# Autodesk Inventor assembly: Reducer_Motor_HG-KR13
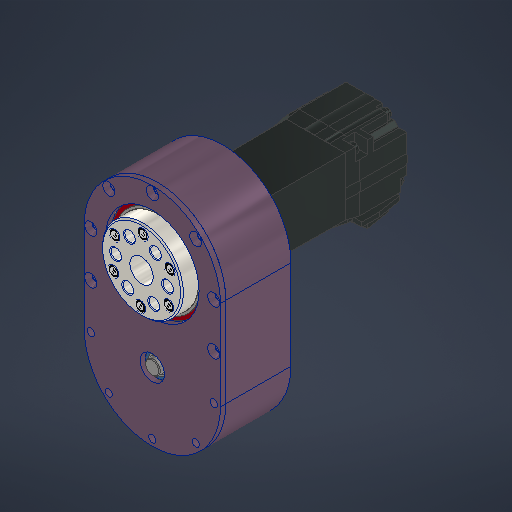
[picture p0: Inventor's stored thumbnail of the model, 512x512]
Saved by Autodesk Inventor 2026 (Build 300175000, 175)
## iProperties
Created: 2025-12-04
Part Number: Reducer_Motor_HG-KR13
Document SubType Name: Assembly
Designer: DanielFGarzon
Mass: 1257.96 g
Surface Area: 1181.01 cm^2
Volume: 298.819 cm^3
Density: 4.20977 g/cm^3
Author: DanielFGarzon
## Documents named in this file (17)
- D:\POLIMI\3RD SEMESTER\Industrial Robotics\Project\Mine\Reducer_02\Reducer_Motor_HG-KR13.iam
- D:\POLIMI\3RD SEMESTER\Industrial Robotics\Project\Mine\Reducer_02\Housing.ipt
- D:\POLIMI\3RD SEMESTER\Industrial Robotics\Project\Mine\Reducer_02\Bearing_08_16_04.ipt
- D:\POLIMI\3RD SEMESTER\Industrial Robotics\Project\Mine\Reducer_02\Bearing_08_26_08.ipt
- D:\POLIMI\3RD SEMESTER\Industrial Robotics\Project\Mine\Reducer_02\Shaft_8mm.ipt
- D:\POLIMI\3RD SEMESTER\Industrial Robotics\Project\Mine\Reducer_02\Motor_HG-KR13.ipt
- D:\POLIMI\3RD SEMESTER\Industrial Robotics\Project\Mine\Reducer_02\Washer_M8_12_0.3.ipt
- D:\POLIMI\3RD SEMESTER\Industrial Robotics\Project\Mine\Reducer_02\Pulley_3M12T_01.ipt
- D:\POLIMI\3RD SEMESTER\Industrial Robotics\Project\Mine\Reducer_02\Washer_M8_10_3.8.ipt
- D:\POLIMI\3RD SEMESTER\Industrial Robotics\Project\Mine\Reducer_02\Pulley_3M60T_01.ipt
- D:\POLIMI\3RD SEMESTER\Industrial Robotics\Project\Mine\Reducer_02\Washer_M8_14_0.5.ipt
- D:\POLIMI\3RD SEMESTER\Industrial Robotics\Project\Mine\Reducer_02\Pulley_3M12T_02.ipt
- D:\POLIMI\3RD SEMESTER\Industrial Robotics\Project\Mine\Reducer_02\Pulley_3M60T_02.ipt
- D:\POLIMI\3RD SEMESTER\Industrial Robotics\Project\Mine\Reducer_02\ActuationDisk.ipt
- D:\POLIMI\3RD SEMESTER\Industrial Robotics\Project\Mine\Reducer_02\Bearing_45_55_06.ipt
- D:\POLIMI\3RD SEMESTER\Industrial Robotics\Project\Mine\Reducer_02\Cover.ipt
- D:\POLIMI\3RD SEMESTER\Industrial Robotics\Project\Mine\Reducer_02\M3_Screw.ipt
## Components (23 placed, 16 different names)
1. Housing:1 — Mate:1, Mate:2, Flush:1, Mate:4, Mate:5, Mate:6, Mate:45
2. Bearing_08_16_04:1 — Mate:1, Mate:2, Mate:3, Mate:7
3. Bearing_08_26_08:1 — Mate:22, Mate:30, Mate:34, Mate:35
4. Shaft_8mm:1 — Mate:3, Flush:1, Mate:8, Mate:20, Mate:27, Mate:32, Mate:47
5. Motor_HG-KR13:1 — Mate:4, Mate:5, Mate:6, Mate:11, Mate:12, Mate:22, Mate:24, Mate:25, Mate:29
6. Washer_M8_12_0.3:1 — Mate:7, Mate:8, Mate:26
7. Pulley_3M12T_01:1 — Mate:23, Mate:25, Mate:28
8. Washer_M8_10_3.8:1 — Mate:11, Mate:12, Mate:23, Mate:24
9. Pulley_3M60T_01:1 — Mate:26, Mate:27, Mate:33
10. Washer_M8_14_0.5:1 — Mate:28, Mate:29, Mate:30
11. Washer_M8_14_0.5:2 — Mate:20, Mate:31, Mate:33
12. Pulley_3M12T_02:1 — Mate:31, Mate:32
13. Pulley_3M60T_02:1 — Mate:34, Mate:35, Mate:40, Mate:41, Mate:42
14. ActuationDisk:1 — Mate:40, Mate:41, Mate:42, Mate:43, Mate:44, Mate:46, Mate:50, Mate:51, Mate:52, Mate:53, Mate:54, Mate:55, Flush:2, Flush:3, Flush:4, Flush:5, Flush:6, Flush:7
15. Bearing_45_55_06:1 — Mate:43, Mate:44
16. Cover:1 — Mate:45, Mate:46, Mate:47, Mate:48, Mate:49
17. Bearing_08_16_04:3 — Mate:48, Mate:49
18. M3_Screw:1 — Mate:51, Flush:3
19. M3_Screw:2 — Mate:55, Flush:6
20. M3_Screw:3 — Mate:54, Flush:5
21. M3_Screw:4 — Mate:50, Flush:2
22. M3_Screw:5 — Mate:52, Flush:4
23. M3_Screw:6 — Mate:53, Flush:7
## Relationships (48: Mate 41, Flush 7)
- Mate:1: Housing:1 ↔ Bearing_08_16_04:1
- Mate:2: Housing:1 ↔ Bearing_08_16_04:1
- Mate:3: Bearing_08_16_04:1 ↔ Shaft_8mm:1
- Flush:1: Housing:1 ↔ Shaft_8mm:1
- Mate:4: Housing:1 ↔ Motor_HG-KR13:1
- Mate:5: Housing:1 ↔ Motor_HG-KR13:1
- Mate:6: Housing:1 ↔ Motor_HG-KR13:1
- Mate:7: Bearing_08_16_04:1 ↔ Washer_M8_12_0.3:1
- Mate:8: Shaft_8mm:1 ↔ Washer_M8_12_0.3:1
- Mate:11: Motor_HG-KR13:1 ↔ Washer_M8_10_3.8:1
- Mate:12: Motor_HG-KR13:1 ↔ Washer_M8_10_3.8:1
- Mate:20: Shaft_8mm:1 ↔ Washer_M8_14_0.5:2
- Mate:22: Bearing_08_26_08:1 ↔ Motor_HG-KR13:1
- Mate:23: Pulley_3M12T_01:1 ↔ Washer_M8_10_3.8:1
- Mate:24: Motor_HG-KR13:1 ↔ Washer_M8_10_3.8:1
- Mate:25: Motor_HG-KR13:1 ↔ Pulley_3M12T_01:1
- Mate:26: Washer_M8_12_0.3:1 ↔ Pulley_3M60T_01:1
- Mate:27: Shaft_8mm:1 ↔ Pulley_3M60T_01:1
- Mate:28: Pulley_3M12T_01:1 ↔ Washer_M8_14_0.5:1
- Mate:29: Motor_HG-KR13:1 ↔ Washer_M8_14_0.5:1
- Mate:30: Bearing_08_26_08:1 ↔ Washer_M8_14_0.5:1
- Mate:31: Washer_M8_14_0.5:2 ↔ Pulley_3M12T_02:1
- Mate:32: Shaft_8mm:1 ↔ Pulley_3M12T_02:1
- Mate:33: Pulley_3M60T_01:1 ↔ Washer_M8_14_0.5:2
- Mate:34: Bearing_08_26_08:1 ↔ Pulley_3M60T_02:1
- Mate:35: Bearing_08_26_08:1 ↔ Pulley_3M60T_02:1
- Mate:40: Pulley_3M60T_02:1 ↔ ActuationDisk:1
- Mate:41: Pulley_3M60T_02:1 ↔ ActuationDisk:1
- Mate:42: Pulley_3M60T_02:1 ↔ ActuationDisk:1
- Mate:43: ActuationDisk:1 ↔ Bearing_45_55_06:1
- Mate:44: ActuationDisk:1 ↔ Bearing_45_55_06:1
- Mate:45: Housing:1 ↔ Cover:1
- Mate:46: ActuationDisk:1 ↔ Cover:1
- Mate:47: Shaft_8mm:1 ↔ Cover:1
- Mate:48: Cover:1 ↔ Bearing_08_16_04:3
- Mate:49: Cover:1 ↔ Bearing_08_16_04:3
- Mate:50: ActuationDisk:1 ↔ M3_Screw:4
- Mate:51: ActuationDisk:1 ↔ M3_Screw:1
- Mate:52: ActuationDisk:1 ↔ M3_Screw:5
- Mate:53: ActuationDisk:1 ↔ M3_Screw:6
- Mate:54: ActuationDisk:1 ↔ M3_Screw:3
- Mate:55: ActuationDisk:1 ↔ M3_Screw:2
- Flush:2: ActuationDisk:1 ↔ M3_Screw:4
- Flush:3: ActuationDisk:1 ↔ M3_Screw:1
- Flush:4: ActuationDisk:1 ↔ M3_Screw:5
- Flush:5: ActuationDisk:1 ↔ M3_Screw:3
- Flush:6: ActuationDisk:1 ↔ M3_Screw:2
- Flush:7: ActuationDisk:1 ↔ M3_Screw:6
